# Autodesk Inventor assembly: Assembly1
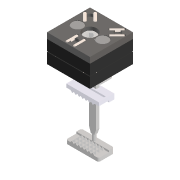
[picture p0: Inventor's stored thumbnail of the model, 180x180]
Saved by Autodesk Inventor 2019 (Build 230136000, 136)
## iProperties
Created: 2021-09-08
Part Number: Assembly1
Document SubType Name: Assembly
Designer: Nikita
Author: Nikita
## Documents named in this file (6)
- C:\Users\nvladi\Documents\Inventor\mesoSPIM_design_benchtop_V2\mesoSPIM\sample_handling\IDISCO-Sampleholder\Clamp-assembly.iam
- C:\Users\nvladi\Documents\Inventor\mesoSPIM_design_benchtop_V2\mesoSPIM\sample_handling\IDISCO-Sampleholder\gravity-clamp-base9x19mm-part1.ipt
- C:\Users\nvladi\Documents\Inventor\mesoSPIM_design_benchtop_V2\mesoSPIM\sample_handling\IDISCO-Sampleholder\gravity-clamp-base9x19mm-part2(moving).ipt
- C:\Users\nvladi\Documents\Inventor\mesoSPIM_design_benchtop_V2\library\Thorlabs\kinematic_bases\KB25_M-Step.ipt
- C:\Users\nvladi\Documents\Inventor\mesoSPIM_design_benchtop_V2\library\Thorlabs\kinematic_bases\KBT25_bottom_vgroove_simplified.ipt
- C:\Users\nvladi\Documents\Inventor\mesoSPIM_design_benchtop_V2\library\Thorlabs\other\screwM4-12mm.ipt
## Components (5 placed, 5 different names)
1. gravity-clamp-base9x19mm-part1:1 — Mate:1, Insert:1, Mate:2, Mate:3, Insert:2
2. gravity-clamp-base9x19mm-part2(moving):3 — Mate:1, Mate:2, Mate:3
3. KB25_M-Step:1 — Insert:1
4. KBT25_bottom_vgroove_simplified:1 — Insert:2, Insert:3
5. screwM4-12mm:1 — Insert:3
## Relationships (6: Mate 3, Insert 3)
- Mate:1: gravity-clamp-base9x19mm-part1:1 ↔ gravity-clamp-base9x19mm-part2(moving):3
- Insert:1: gravity-clamp-base9x19mm-part1:1 ↔ KB25_M-Step:1
- Mate:2: gravity-clamp-base9x19mm-part1:1 ↔ gravity-clamp-base9x19mm-part2(moving):3
- Mate:3: gravity-clamp-base9x19mm-part1:1 ↔ gravity-clamp-base9x19mm-part2(moving):3
- Insert:2 (10 mm): gravity-clamp-base9x19mm-part1:1 ↔ KBT25_bottom_vgroove_simplified:1
- Insert:3 (5 mm): KBT25_bottom_vgroove_simplified:1 ↔ screwM4-12mm:1
